# Autodesk Inventor assembly: Assembly1
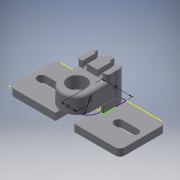
[picture p0: Inventor's stored thumbnail of the model, 180x180]
Saved by Autodesk Inventor 2016 (Build 200138000, 138)
## iProperties
Created: 2016-02-21
Part Number: Assembly1
Document SubType Name: Assembly
Designer: Mikkel
Author: Mikkel
## Documents named in this file (3)
- D:\OneDrive\Til NAS\Projekter\Inventor\3D-projects\Misc-vitamins\Opar-jhead-mount\Assembly1.iam
- D:\OneDrive\Til NAS\Projekter\Inventor\3D-projects\Misc-vitamins\Opar-jhead-mount\plate.ipt
- D:\OneDrive\Til NAS\Projekter\Inventor\3D-projects\Misc-vitamins\Opar-jhead-mount\clip.ipt
## Components (2 placed, 2 different names)
1. plate:1 — Flush:1, Flush:2
2. clip:1 — Flush:1, Flush:2
## Relationships (2: Flush 2)
- Flush:1: plate:1 ↔ clip:1
- Flush:2: plate:1 ↔ clip:1
